# Autodesk Inventor assembly: Assieme2
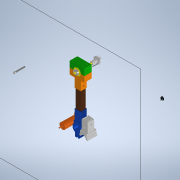
[picture p0: Inventor's stored thumbnail of the model, 180x180]
Saved by Autodesk Inventor 2020 (Build 240168000, 168)
## iProperties
Created: 2019-10-11
Part Number: Assieme2
Document SubType Name: Assembly
Designer: socci
Author: socci
## Documents named in this file (16)
- C:\Users\socci\Desktop\mv-Project\04_PartDraw\Modello_3D.iam
- C:\Users\socci\Desktop\mv-Project\04_PartDraw\Componenti\1_Asse_cuscinetti.ipt
- C:\Users\socci\Desktop\mv-Project\04_PartDraw\Componenti\2_Connettore_inf_sup.ipt
- C:\Users\socci\Desktop\mv-Project\04_PartDraw\Componenti\3_Connettore_inf_INF.ipt
- C:\Users\socci\Desktop\mv-Project\04_PartDraw\Componenti\4_barra.ipt
- C:\Users\socci\Desktop\mv-Project\04_PartDraw\Componenti\5_Connettore_sup_inf.ipt
- C:\Users\socci\Desktop\mv-Project\04_PartDraw\Componenti\6_Vite_M5_L40.ipt
- C:\Users\socci\Desktop\mv-Project\04_PartDraw\Componenti\7_Motore.ipt
- C:\Users\socci\Desktop\mv-Project\04_PartDraw\Componenti\8_Connettore_sup.ipt
- C:\Users\socci\Desktop\mv-Project\04_PartDraw\Componenti\9_Flangia.ipt
- C:\Users\socci\Desktop\mv-Project\04_PartDraw\Componenti\10_MPU_6050.ipt
- C:\Users\socci\Desktop\mv-Project\04_PartDraw\Componenti\11_Connettore_MPU.ipt
- C:\Users\socci\Desktop\mv-Project\04_PartDraw\Componenti\12_Vite_M3_L30.ipt
- C:\Users\socci\Documents\13_Dado_M3.ipt
- C:\Users\socci\Documents\Inventor\Content Center Files\R2020\it-IT\Bearing GB_T 5800-2003\Rolling bearing GB_T 5800-2003 -626.ipt
- C:\Users\socci\Documents\Inventor\Content Center Files\R2020\it-IT\AS 1427(05)\AS 1427 - M4 x 40(5) II.ipt
## Components (23 placed, 15 different names)
1. 1_Asse_cuscinetti:1 — Inserimento:1, Inserimento:2, Inserimento:3, Coincidente:12, Coincidente:13, Coincidente:14, Coincidente:15
2. 2_Connettore_inf_sup:1 — Inserimento:1, Coincidente:6, Coincidente:7, Coincidente:8, Inserimento:14, Inserimento:15, Inserimento:16, Inserimento:17
3. 3_Connettore_inf_INF:1 — Inserimento:2
4. 4_barra:1 — Coincidente:6, Coincidente:7, Coincidente:8, Coincidente:9, Coincidente:10, Coincidente:11
5. 5_Connettore_sup_inf:1 — Coincidente:9, Coincidente:10, Coincidente:11
6. 6_Vite_M5_L40:1
7. 7_Motore:1
8. 8_Connettore_sup:1
9. 9_Flangia:1
10. 10_MPU_6050:1 — Inserimento:4, Inserimento:5, Inserimento:6, Inserimento:7
11. 11_Connettore_MPU:1 — Inserimento:3, Inserimento:11, Inserimento:12, Inserimento:13
12. 12_Vite_M3_L30:1 — Inserimento:4
13. 12_Vite_M3_L30:2 — Inserimento:5
14. 13_Dado_M3:1 — Inserimento:6, Inserimento:13
15. 13_Dado_M3:2 — Inserimento:11
16. 13_Dado_M3:3 — Inserimento:7, Inserimento:12
17. 13_Dado_M3:4
18. Bearing GB/T 5800-2003 626:1 — Coincidente:12, Coincidente:14
19. Bearing GB/T 5800-2003 626:2 — Coincidente:13, Coincidente:15
20. AS 1427 H - Metrico M4 x 40:1 — Inserimento:14
21. AS 1427 H - Metrico M4 x 40:2 — Inserimento:15
22. AS 1427 H - Metrico M4 x 40:3 — Inserimento:16
23. AS 1427 H - Metrico M4 x 40:4 — Inserimento:17
## Relationships (24: Insert 14, Mate 10)
- Inserimento:1: 1_Asse_cuscinetti:1 ↔ 2_Connettore_inf_sup:1
- Inserimento:2: 1_Asse_cuscinetti:1 ↔ 3_Connettore_inf_INF:1
- Coincidente:6 [Mate]: 2_Connettore_inf_sup:1 ↔ 4_barra:1
- Coincidente:7 [Mate]: 2_Connettore_inf_sup:1 ↔ 4_barra:1
- Coincidente:8 [Mate]: 2_Connettore_inf_sup:1 ↔ 4_barra:1
- Coincidente:9 [Mate]: 4_barra:1 ↔ 5_Connettore_sup_inf:1
- Coincidente:10 [Mate]: 4_barra:1 ↔ 5_Connettore_sup_inf:1
- Coincidente:11 [Mate]: 4_barra:1 ↔ 5_Connettore_sup_inf:1
- Inserimento:3: 1_Asse_cuscinetti:1 ↔ 11_Connettore_MPU:1
- Inserimento:4: 10_MPU_6050:1 ↔ 12_Vite_M3_L30:1
- Inserimento:5: 10_MPU_6050:1 ↔ 12_Vite_M3_L30:2
- Inserimento:6: 10_MPU_6050:1 ↔ 13_Dado_M3:1
- Inserimento:7: 10_MPU_6050:1 ↔ 13_Dado_M3:3
- Inserimento:11: 11_Connettore_MPU:1 ↔ 13_Dado_M3:2
- Inserimento:12: 11_Connettore_MPU:1 ↔ 13_Dado_M3:3
- Inserimento:13: 11_Connettore_MPU:1 ↔ 13_Dado_M3:1
- Coincidente:12 [Mate]: 1_Asse_cuscinetti:1 ↔ Bearing GB/T 5800-2003 626:1
- Coincidente:13 [Mate]: 1_Asse_cuscinetti:1 ↔ Bearing GB/T 5800-2003 626:2
- Coincidente:14 [Mate] (2.5 mm): 1_Asse_cuscinetti:1 ↔ Bearing GB/T 5800-2003 626:1
- Coincidente:15 [Mate] (1.5 mm): 1_Asse_cuscinetti:1 ↔ Bearing GB/T 5800-2003 626:2
- Inserimento:14: 2_Connettore_inf_sup:1 ↔ AS 1427 H - Metrico M4 x 40:1
- Inserimento:15: 2_Connettore_inf_sup:1 ↔ AS 1427 H - Metrico M4 x 40:2
- Inserimento:16: 2_Connettore_inf_sup:1 ↔ AS 1427 H - Metrico M4 x 40:3
- Inserimento:17: 2_Connettore_inf_sup:1 ↔ AS 1427 H - Metrico M4 x 40:4
